# Autodesk Inventor assembly: 08-03-00-000_TurnGTElectronics
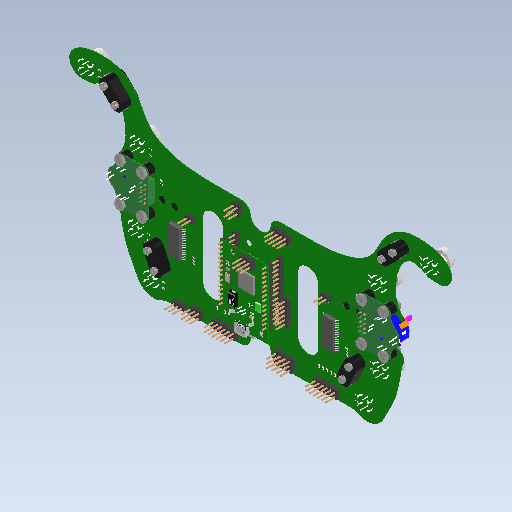
[picture p0: Inventor's stored thumbnail of the model, 512x512]
Saved by Autodesk Inventor 2020 (Build 240168000, 168)
## iProperties
Created: 2021-07-25
Part Number: 08-03-00-000_TurnGTElectronics
Document SubType Name: Assembly
Designer: Eric
Mass: 25.2475 g
Surface Area: 546.628 cm^2
Volume: 21.4632 cm^3
Density: 1.17631 g/cm^3
Author: Eric
## Documents named in this file (13)
- C:\Users\Eric\Documents\repos\DIY_CAD_WheelButtonPlate\CAD\Inventor\08-03-00-000_TurnGTElectronics.iam
- C:\Users\Eric\Documents\repos\DIY_CAD_WheelButtonPlate\CAD\Inventor\08-03-01-001_turnRacingMain.ipt
- C:\Users\Eric\Documents\repos\DIY_CAD_WheelButtonPlate\CAD\Inventor\08-03-01-002_arduinoOwnarduinoLeonardoOwn.ipt
- C:\Users\Eric\Documents\repos\DIY_CAD_WheelButtonPlate\CAD\Inventor\08-03-01-003_funkyDaugtherBoard.ipt
- C:\Users\Eric\Documents\repos\DIY_CAD_WheelButtonPlate\CAD\Inventor\08-03-02-004_buttonCap.ipt
- C:\Users\Eric\Documents\repos\DIY_CAD_WheelButtonPlate\CAD\Inventor\08-02-01-007_centerPCBSpacer.ipt
- C:\Users\Eric\Documents\repos\DIY_CAD_WheelButtonPlate\CAD\Inventor\08-02-01-006_PCBSpacer.ipt
- C:\Users\Eric\Documents\repos\DIY_CAD_WheelButtonPlate\CAD\Inventor\08-02-01-008_funkySwitchSpacer.ipt
- C:\Users\Eric\Documents\repos\DIY_CAD_WheelButtonPlate\CAD\Inventor\08-02-01-009_fixPCBSpacer.ipt
- C:\Users\Eric\Documents\Inventor\Content Center Files\R2020\de-DE\DIN 439-2\DIN 439 - M2 x 0,4.ipt
- C:\Users\Eric\Documents\Inventor\Content Center Files\R2020\de-DE\ISO 4762(1)\DIN EN ISO 4762 - M2 x 10.ipt
- C:\Users\Eric\Documents\Inventor\Content Center Files\R2020\de-DE\ISO 4762(1)\DIN EN ISO 4762 - M3 x 8.ipt
- C:\Users\Eric\Documents\Inventor\Content Center Files\R2020\de-DE\ISO 4032(1)\ISO 4032 - M3DIN EN.ipt
## Components (62 placed, 12 different names)
1. 08-03-01-002_arduinoOwnarduinoLeonardoOwn:1 — Passend:1, Passend:2, Passend:3
2. 08-03-01-001_turnRacingMain:1 — Passend:1, Passend:2, Passend:3, Passend:4, Passend:5, Passend:6, Passend:7, Passend:8, Passend:9, Passend:10, Passend:12, Passend:13, Passend:14, Passend:15, Passend:16, Passend:17, Passend:18, Passend:19, Passend:20, Passend:21, Passend:22, Passend:23, Passend:24, Passend:25, Passend:26, Passend:27, Passend:28, Passend:29, Passend:30, Passend:31, Passend:32, Passend:33, Passend:34, Passend:35, Passend:36, Passend:37, Passend:38, Passend:39, Passend:40, Passend:41, Passend:42, Passend:43, Passend:44, Passend:45, Passend:46, Passend:47, Passend:48, Passend:49, Passend:50, Passend:51, Passend:52, Passend:53, Passend:54, Passend:55, Passend:56, Passend:57, Passend:58, Passend:59, Passend:60, Fluchtend:1, Fluchtend:2, Fluchtend:3, Fluchtend:4, Einfügen:9, Einfügen:10, Einfügen:11, Einfügen:12, Einfügen:13, Einfügen:14, Einfügen:15, Einfügen:16
3. 08-03-01-003_funkyDaugtherBoard:1 — Passend:4, Passend:6, Passend:7, Einfügen:17, Einfügen:18, Einfügen:19, Einfügen:20
4. 08-03-01-003_funkyDaugtherBoard:2 — Passend:5, Passend:8, Passend:9, Einfügen:21, Einfügen:22, Einfügen:23, Einfügen:24
5. 08-03-02-004_buttonCap:1 — Passend:10, Passend:12
6. 08-03-02-004_buttonCap:2 — Passend:15, Passend:24
7. 08-03-02-004_buttonCap:3 — Passend:14, Passend:25
8. 08-03-02-004_buttonCap:4 — Passend:13, Passend:26
9. 08-03-02-004_buttonCap:5 — Passend:19, Passend:23
10. 08-03-02-004_buttonCap:6 — Passend:17, Passend:21
11. 08-03-02-004_buttonCap:7 — Passend:16, Passend:20
12. 08-03-02-004_buttonCap:8 — Passend:18, Passend:22
13. 08-02-01-007_centerPCBSpacer:1 — Passend:42, Passend:43, Passend:44
14. 08-02-01-007_centerPCBSpacer:2 — Passend:39, Passend:40, Passend:41
15. 08-02-01-006_PCBSpacer:1 — Passend:27, Passend:35, Passend:36, Passend:61, Passend:62, Passend:83, Passend:84, Passend:85, Passend:86
16. 08-02-01-006_PCBSpacer:2 — Passend:28, Passend:37, Passend:38, Passend:63, Passend:64, Passend:79, Passend:82, Passend:87, Passend:88
17. 08-02-01-006_PCBSpacer:3 — Passend:29, Passend:33, Passend:34, Passend:67, Passend:68, Passend:77, Passend:78, Passend:89, Passend:90
18. 08-02-01-006_PCBSpacer:4 — Passend:30, Passend:31, Passend:32, Passend:65, Passend:66, Passend:80, Passend:81, Passend:91, Passend:92
19. 08-02-01-008_funkySwitchSpacer:1 — Passend:55, Passend:57
20. 08-02-01-008_funkySwitchSpacer:2 — Passend:46, Passend:47
21. 08-02-01-008_funkySwitchSpacer:3 — Passend:54, Passend:59
22. 08-02-01-008_funkySwitchSpacer:4 — Passend:45, Passend:52
23. 08-02-01-008_funkySwitchSpacer:5 — Passend:53, Passend:60
24. 08-02-01-008_funkySwitchSpacer:6 — Passend:56, Passend:58
25. 08-02-01-008_funkySwitchSpacer:7 — Passend:50, Passend:51
26. 08-02-01-008_funkySwitchSpacer:8 — Passend:48, Passend:49
27. 08-02-01-009_fixPCBSpacer:1 — Fluchtend:1, Passend:67, Passend:68, Passend:71, Passend:72, Einfügen:5, Einfügen:6
28. 08-02-01-009_fixPCBSpacer:2 — Fluchtend:2, Passend:65, Passend:66, Passend:69, Passend:70, Einfügen:7, Einfügen:8
29. 08-02-01-009_fixPCBSpacer:3 — Fluchtend:3, Passend:63, Passend:64, Passend:75, Passend:76, Einfügen:1, Einfügen:2
30. 08-02-01-009_fixPCBSpacer:4 — Fluchtend:4, Passend:61, Passend:62, Passend:73, Passend:74, Einfügen:3, Einfügen:4
31. DIN 439-2 - ersetzt durch DIN EN 24035/28675 M2:1 — Passend:69, Passend:80, Passend:92
32. DIN 439-2 - ersetzt durch DIN EN 24035/28675 M2:2 — Passend:75, Passend:82, Passend:88
33. DIN 439-2 - ersetzt durch DIN EN 24035/28675 M2:3 — Passend:76, Passend:79, Passend:87
34. DIN 439-2 - ersetzt durch DIN EN 24035/28675 M2:4 — Passend:74, Passend:83, Passend:86
35. DIN 439-2 - ersetzt durch DIN EN 24035/28675 M2:5 — Passend:70, Passend:81, Passend:91
36. DIN 439-2 - ersetzt durch DIN EN 24035/28675 M2:6 — Passend:71, Passend:78, Passend:89
37. DIN 439-2 - ersetzt durch DIN EN 24035/28675 M2:7 — Passend:72, Passend:77, Passend:90
38. DIN 439-2 - ersetzt durch DIN EN 24035/28675 M2:8 — Passend:73, Passend:84, Passend:85
39. DIN EN ISO 4762 M2 x 10:1 — Einfügen:7
40. DIN EN ISO 4762 M2 x 10:2 — Einfügen:8
41. DIN EN ISO 4762 M2 x 10:3 — Einfügen:5
42. DIN EN ISO 4762 M2 x 10:4 — Einfügen:6
43. DIN EN ISO 4762 M2 x 10:5 — Einfügen:4
44. DIN EN ISO 4762 M2 x 10:6 — Einfügen:3
45. DIN EN ISO 4762 M2 x 10:7 — Einfügen:2
46. DIN EN ISO 4762 M2 x 10:8 — Einfügen:1
47. DIN EN ISO 4762 M3 x 8:1 — Einfügen:9
48. DIN EN ISO 4762 M3 x 8:2 — Einfügen:10
49. DIN EN ISO 4762 M3 x 8:3 — Einfügen:11
50. DIN EN ISO 4762 M3 x 8:4 — Einfügen:12
51. DIN EN ISO 4762 M3 x 8:5 — Einfügen:13
52. DIN EN ISO 4762 M3 x 8:6 — Einfügen:14
53. DIN EN ISO 4762 M3 x 8:7 — Einfügen:15
54. DIN EN ISO 4762 M3 x 8:8 — Einfügen:16
55. DIN EN 24032 M3:1 — Einfügen:17
56. DIN EN 24032 M3:2 — Einfügen:18
57. DIN EN 24032 M3:3 — Einfügen:19
58. DIN EN 24032 M3:4 — Einfügen:20
59. DIN EN 24032 M3:5 — Einfügen:21
60. DIN EN 24032 M3:6 — Einfügen:22
61. DIN EN 24032 M3:7 — Einfügen:23
62. DIN EN 24032 M3:8 — Einfügen:24
## Relationships (119: Mate 91, Insert 24, Flush 4)
- Passend:1 [Mate]: 08-03-01-002_arduinoOwnarduinoLeonardoOwn:1 ↔ 08-03-01-001_turnRacingMain:1
- Passend:2 [Mate]: 08-03-01-002_arduinoOwnarduinoLeonardoOwn:1 ↔ 08-03-01-001_turnRacingMain:1
- Passend:3 [Mate] (10 mm): 08-03-01-002_arduinoOwnarduinoLeonardoOwn:1 ↔ 08-03-01-001_turnRacingMain:1
- Passend:4 [Mate] (4 mm): 08-03-01-001_turnRacingMain:1 ↔ 08-03-01-003_funkyDaugtherBoard:1
- Passend:5 [Mate] (4 mm): 08-03-01-001_turnRacingMain:1 ↔ 08-03-01-003_funkyDaugtherBoard:2
- Passend:6 [Mate]: 08-03-01-001_turnRacingMain:1 ↔ 08-03-01-003_funkyDaugtherBoard:1
- Passend:7 [Mate]: 08-03-01-001_turnRacingMain:1 ↔ 08-03-01-003_funkyDaugtherBoard:1
- Passend:8 [Mate]: 08-03-01-001_turnRacingMain:1 ↔ 08-03-01-003_funkyDaugtherBoard:2
- Passend:9 [Mate]: 08-03-01-001_turnRacingMain:1 ↔ 08-03-01-003_funkyDaugtherBoard:2
- Passend:10 [Mate]: 08-03-01-001_turnRacingMain:1 ↔ 08-03-02-004_buttonCap:1
- Passend:12 [Mate]: 08-03-01-001_turnRacingMain:1 ↔ 08-03-02-004_buttonCap:1
- Passend:13 [Mate]: 08-03-01-001_turnRacingMain:1 ↔ 08-03-02-004_buttonCap:4
- Passend:14 [Mate]: 08-03-01-001_turnRacingMain:1 ↔ 08-03-02-004_buttonCap:3
- Passend:15 [Mate]: 08-03-01-001_turnRacingMain:1 ↔ 08-03-02-004_buttonCap:2
- Passend:16 [Mate]: 08-03-01-001_turnRacingMain:1 ↔ 08-03-02-004_buttonCap:7
- Passend:17 [Mate]: 08-03-01-001_turnRacingMain:1 ↔ 08-03-02-004_buttonCap:6
- Passend:18 [Mate]: 08-03-01-001_turnRacingMain:1 ↔ 08-03-02-004_buttonCap:8
- Passend:19 [Mate]: 08-03-01-001_turnRacingMain:1 ↔ 08-03-02-004_buttonCap:5
- Passend:20 [Mate]: 08-03-01-001_turnRacingMain:1 ↔ 08-03-02-004_buttonCap:7
- Passend:21 [Mate]: 08-03-01-001_turnRacingMain:1 ↔ 08-03-02-004_buttonCap:6
- Passend:22 [Mate]: 08-03-01-001_turnRacingMain:1 ↔ 08-03-02-004_buttonCap:8
- Passend:23 [Mate]: 08-03-01-001_turnRacingMain:1 ↔ 08-03-02-004_buttonCap:5
- Passend:24 [Mate]: 08-03-01-001_turnRacingMain:1 ↔ 08-03-02-004_buttonCap:2
- Passend:25 [Mate]: 08-03-01-001_turnRacingMain:1 ↔ 08-03-02-004_buttonCap:3
- Passend:26 [Mate]: 08-03-01-001_turnRacingMain:1 ↔ 08-03-02-004_buttonCap:4
- Passend:27 [Mate]: 08-03-01-001_turnRacingMain:1 ↔ 08-02-01-006_PCBSpacer:1
- Passend:28 [Mate]: 08-03-01-001_turnRacingMain:1 ↔ 08-02-01-006_PCBSpacer:2
- Passend:29 [Mate]: 08-03-01-001_turnRacingMain:1 ↔ 08-02-01-006_PCBSpacer:3
- Passend:30 [Mate]: 08-03-01-001_turnRacingMain:1 ↔ 08-02-01-006_PCBSpacer:4
- Passend:31 [Mate]: 08-03-01-001_turnRacingMain:1 ↔ 08-02-01-006_PCBSpacer:4
- Passend:32 [Mate]: 08-03-01-001_turnRacingMain:1 ↔ 08-02-01-006_PCBSpacer:4
- Passend:33 [Mate]: 08-03-01-001_turnRacingMain:1 ↔ 08-02-01-006_PCBSpacer:3
- Passend:34 [Mate]: 08-03-01-001_turnRacingMain:1 ↔ 08-02-01-006_PCBSpacer:3
- Passend:35 [Mate]: 08-03-01-001_turnRacingMain:1 ↔ 08-02-01-006_PCBSpacer:1
- Passend:36 [Mate]: 08-03-01-001_turnRacingMain:1 ↔ 08-02-01-006_PCBSpacer:1
- Passend:37 [Mate]: 08-03-01-001_turnRacingMain:1 ↔ 08-02-01-006_PCBSpacer:2
- Passend:38 [Mate]: 08-03-01-001_turnRacingMain:1 ↔ 08-02-01-006_PCBSpacer:2
- Passend:39 [Mate]: 08-03-01-001_turnRacingMain:1 ↔ 08-02-01-007_centerPCBSpacer:2
- Passend:40 [Mate]: 08-03-01-001_turnRacingMain:1 ↔ 08-02-01-007_centerPCBSpacer:2
- Passend:41 [Mate]: 08-03-01-001_turnRacingMain:1 ↔ 08-02-01-007_centerPCBSpacer:2
- Passend:42 [Mate]: 08-03-01-001_turnRacingMain:1 ↔ 08-02-01-007_centerPCBSpacer:1
- Passend:43 [Mate]: 08-03-01-001_turnRacingMain:1 ↔ 08-02-01-007_centerPCBSpacer:1
- Passend:44 [Mate]: 08-03-01-001_turnRacingMain:1 ↔ 08-02-01-007_centerPCBSpacer:1
- Passend:45 [Mate]: 08-03-01-001_turnRacingMain:1 ↔ 08-02-01-008_funkySwitchSpacer:4
- Passend:46 [Mate]: 08-03-01-001_turnRacingMain:1 ↔ 08-02-01-008_funkySwitchSpacer:2
- Passend:47 [Mate]: 08-03-01-001_turnRacingMain:1 ↔ 08-02-01-008_funkySwitchSpacer:2
- Passend:48 [Mate]: 08-03-01-001_turnRacingMain:1 ↔ 08-02-01-008_funkySwitchSpacer:8
- Passend:49 [Mate]: 08-03-01-001_turnRacingMain:1 ↔ 08-02-01-008_funkySwitchSpacer:8
- Passend:50 [Mate]: 08-03-01-001_turnRacingMain:1 ↔ 08-02-01-008_funkySwitchSpacer:7
- Passend:51 [Mate]: 08-03-01-001_turnRacingMain:1 ↔ 08-02-01-008_funkySwitchSpacer:7
- Passend:52 [Mate]: 08-03-01-001_turnRacingMain:1 ↔ 08-02-01-008_funkySwitchSpacer:4
- Passend:53 [Mate]: 08-03-01-001_turnRacingMain:1 ↔ 08-02-01-008_funkySwitchSpacer:5
- Passend:54 [Mate]: 08-03-01-001_turnRacingMain:1 ↔ 08-02-01-008_funkySwitchSpacer:3
- Passend:55 [Mate]: 08-03-01-001_turnRacingMain:1 ↔ 08-02-01-008_funkySwitchSpacer:1
- Passend:56 [Mate]: 08-03-01-001_turnRacingMain:1 ↔ 08-02-01-008_funkySwitchSpacer:6
- Passend:57 [Mate]: 08-03-01-001_turnRacingMain:1 ↔ 08-02-01-008_funkySwitchSpacer:1
- Passend:58 [Mate]: 08-03-01-001_turnRacingMain:1 ↔ 08-02-01-008_funkySwitchSpacer:6
- Passend:59 [Mate]: 08-03-01-001_turnRacingMain:1 ↔ 08-02-01-008_funkySwitchSpacer:3
- Passend:60 [Mate]: 08-03-01-001_turnRacingMain:1 ↔ 08-02-01-008_funkySwitchSpacer:5
- Fluchtend:1 [Flush] (1.6 mm): 08-03-01-001_turnRacingMain:1 ↔ 08-02-01-009_fixPCBSpacer:1
- Fluchtend:2 [Flush] (1.6 mm): 08-03-01-001_turnRacingMain:1 ↔ 08-02-01-009_fixPCBSpacer:2
- Fluchtend:3 [Flush] (1.6 mm): 08-03-01-001_turnRacingMain:1 ↔ 08-02-01-009_fixPCBSpacer:3
- Fluchtend:4 [Flush] (1.6 mm): 08-03-01-001_turnRacingMain:1 ↔ 08-02-01-009_fixPCBSpacer:4
- Passend:61 [Mate]: 08-02-01-006_PCBSpacer:1 ↔ 08-02-01-009_fixPCBSpacer:4
- Passend:62 [Mate]: 08-02-01-006_PCBSpacer:1 ↔ 08-02-01-009_fixPCBSpacer:4
- Passend:63 [Mate]: 08-02-01-006_PCBSpacer:2 ↔ 08-02-01-009_fixPCBSpacer:3
- Passend:64 [Mate]: 08-02-01-006_PCBSpacer:2 ↔ 08-02-01-009_fixPCBSpacer:3
- Passend:65 [Mate]: 08-02-01-006_PCBSpacer:4 ↔ 08-02-01-009_fixPCBSpacer:2
- Passend:66 [Mate]: 08-02-01-006_PCBSpacer:4 ↔ 08-02-01-009_fixPCBSpacer:2
- Passend:67 [Mate]: 08-02-01-006_PCBSpacer:3 ↔ 08-02-01-009_fixPCBSpacer:1
- Passend:68 [Mate]: 08-02-01-006_PCBSpacer:3 ↔ 08-02-01-009_fixPCBSpacer:1
- Passend:69 [Mate]: 08-02-01-009_fixPCBSpacer:2 ↔ DIN 439-2 - ersetzt durch DIN EN 24035/28675 M2:1
- Passend:70 [Mate]: 08-02-01-009_fixPCBSpacer:2 ↔ DIN 439-2 - ersetzt durch DIN EN 24035/28675 M2:5
- Passend:71 [Mate]: 08-02-01-009_fixPCBSpacer:1 ↔ DIN 439-2 - ersetzt durch DIN EN 24035/28675 M2:6
- Passend:72 [Mate]: 08-02-01-009_fixPCBSpacer:1 ↔ DIN 439-2 - ersetzt durch DIN EN 24035/28675 M2:7
- Passend:73 [Mate]: 08-02-01-009_fixPCBSpacer:4 ↔ DIN 439-2 - ersetzt durch DIN EN 24035/28675 M2:8
- Passend:74 [Mate]: 08-02-01-009_fixPCBSpacer:4 ↔ DIN 439-2 - ersetzt durch DIN EN 24035/28675 M2:4
- Passend:75 [Mate]: 08-02-01-009_fixPCBSpacer:3 ↔ DIN 439-2 - ersetzt durch DIN EN 24035/28675 M2:2
- Passend:76 [Mate]: 08-02-01-009_fixPCBSpacer:3 ↔ DIN 439-2 - ersetzt durch DIN EN 24035/28675 M2:3
- Passend:77 [Mate]: 08-02-01-006_PCBSpacer:3 ↔ DIN 439-2 - ersetzt durch DIN EN 24035/28675 M2:7
- Passend:78 [Mate]: 08-02-01-006_PCBSpacer:3 ↔ DIN 439-2 - ersetzt durch DIN EN 24035/28675 M2:6
- Passend:79 [Mate]: 08-02-01-006_PCBSpacer:2 ↔ DIN 439-2 - ersetzt durch DIN EN 24035/28675 M2:3
- Passend:80 [Mate]: 08-02-01-006_PCBSpacer:4 ↔ DIN 439-2 - ersetzt durch DIN EN 24035/28675 M2:1
- Passend:81 [Mate]: 08-02-01-006_PCBSpacer:4 ↔ DIN 439-2 - ersetzt durch DIN EN 24035/28675 M2:5
- Passend:82 [Mate]: 08-02-01-006_PCBSpacer:2 ↔ DIN 439-2 - ersetzt durch DIN EN 24035/28675 M2:2
- Passend:83 [Mate]: 08-02-01-006_PCBSpacer:1 ↔ DIN 439-2 - ersetzt durch DIN EN 24035/28675 M2:4
- Passend:84 [Mate]: 08-02-01-006_PCBSpacer:1 ↔ DIN 439-2 - ersetzt durch DIN EN 24035/28675 M2:8
- Passend:85 [Mate]: 08-02-01-006_PCBSpacer:1 ↔ DIN 439-2 - ersetzt durch DIN EN 24035/28675 M2:8
- Passend:86 [Mate]: 08-02-01-006_PCBSpacer:1 ↔ DIN 439-2 - ersetzt durch DIN EN 24035/28675 M2:4
- Passend:87 [Mate]: 08-02-01-006_PCBSpacer:2 ↔ DIN 439-2 - ersetzt durch DIN EN 24035/28675 M2:3
- Passend:88 [Mate]: 08-02-01-006_PCBSpacer:2 ↔ DIN 439-2 - ersetzt durch DIN EN 24035/28675 M2:2
- Passend:89 [Mate]: 08-02-01-006_PCBSpacer:3 ↔ DIN 439-2 - ersetzt durch DIN EN 24035/28675 M2:6
- Passend:90 [Mate]: 08-02-01-006_PCBSpacer:3 ↔ DIN 439-2 - ersetzt durch DIN EN 24035/28675 M2:7
- Passend:91 [Mate]: 08-02-01-006_PCBSpacer:4 ↔ DIN 439-2 - ersetzt durch DIN EN 24035/28675 M2:5
- Passend:92 [Mate]: 08-02-01-006_PCBSpacer:4 ↔ DIN 439-2 - ersetzt durch DIN EN 24035/28675 M2:1
- Einfügen:1 [Insert]: 08-02-01-009_fixPCBSpacer:3 ↔ DIN EN ISO 4762 M2 x 10:8
- Einfügen:2 [Insert]: 08-02-01-009_fixPCBSpacer:3 ↔ DIN EN ISO 4762 M2 x 10:7
- Einfügen:3 [Insert]: 08-02-01-009_fixPCBSpacer:4 ↔ DIN EN ISO 4762 M2 x 10:6
- Einfügen:4 [Insert]: 08-02-01-009_fixPCBSpacer:4 ↔ DIN EN ISO 4762 M2 x 10:5
- Einfügen:5 [Insert]: 08-02-01-009_fixPCBSpacer:1 ↔ DIN EN ISO 4762 M2 x 10:3
- Einfügen:6 [Insert]: 08-02-01-009_fixPCBSpacer:1 ↔ DIN EN ISO 4762 M2 x 10:4
- Einfügen:7 [Insert]: 08-02-01-009_fixPCBSpacer:2 ↔ DIN EN ISO 4762 M2 x 10:1
- Einfügen:8 [Insert]: 08-02-01-009_fixPCBSpacer:2 ↔ DIN EN ISO 4762 M2 x 10:2
- Einfügen:9 [Insert]: 08-03-01-001_turnRacingMain:1 ↔ DIN EN ISO 4762 M3 x 8:1
- Einfügen:10 [Insert]: 08-03-01-001_turnRacingMain:1 ↔ DIN EN ISO 4762 M3 x 8:2
- Einfügen:11 [Insert]: 08-03-01-001_turnRacingMain:1 ↔ DIN EN ISO 4762 M3 x 8:3
- Einfügen:12 [Insert]: 08-03-01-001_turnRacingMain:1 ↔ DIN EN ISO 4762 M3 x 8:4
- Einfügen:13 [Insert]: 08-03-01-001_turnRacingMain:1 ↔ DIN EN ISO 4762 M3 x 8:5
- Einfügen:14 [Insert]: 08-03-01-001_turnRacingMain:1 ↔ DIN EN ISO 4762 M3 x 8:6
- Einfügen:15 [Insert]: 08-03-01-001_turnRacingMain:1 ↔ DIN EN ISO 4762 M3 x 8:7
- Einfügen:16 [Insert]: 08-03-01-001_turnRacingMain:1 ↔ DIN EN ISO 4762 M3 x 8:8
- Einfügen:17 [Insert]: 08-03-01-003_funkyDaugtherBoard:1 ↔ DIN EN 24032 M3:1
- Einfügen:18 [Insert]: 08-03-01-003_funkyDaugtherBoard:1 ↔ DIN EN 24032 M3:2
- Einfügen:19 [Insert]: 08-03-01-003_funkyDaugtherBoard:1 ↔ DIN EN 24032 M3:3
- Einfügen:20 [Insert]: 08-03-01-003_funkyDaugtherBoard:1 ↔ DIN EN 24032 M3:4
- Einfügen:21 [Insert]: 08-03-01-003_funkyDaugtherBoard:2 ↔ DIN EN 24032 M3:5
- Einfügen:22 [Insert]: 08-03-01-003_funkyDaugtherBoard:2 ↔ DIN EN 24032 M3:6
- Einfügen:23 [Insert]: 08-03-01-003_funkyDaugtherBoard:2 ↔ DIN EN 24032 M3:7
- Einfügen:24 [Insert]: 08-03-01-003_funkyDaugtherBoard:2 ↔ DIN EN 24032 M3:8
